# Autodesk Inventor assembly: ChainWheelSubAssembly
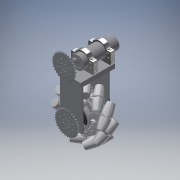
[picture p0: Inventor's stored thumbnail of the model, 180x180]
Saved by Autodesk Inventor 2017 (Build 210142000, 142)
## iProperties
Created: 2017-11-22
Part Number: ChainWheelSubAssembly
Document SubType Name: Assembly
Designer: User
Author: User
## Documents named in this file (9)
- C:\Robotics\CAD\2017-18_CAD\Prototypes\ChainWheelSubAssembly.iam
- C:\Robotics\CAD\COTSParts\Tetrix\tetrix-motor-mounts-1.snapshot.1\Tetrex 2pc motor mount.ipt
- C:\Robotics\CAD\COTSParts\Motors\Andymark 2964  NeveRest 40 Motor.ipt
- C:\Robotics\CAD\COTSParts\Actobotics\545 parts\545618 clamping hub.ipt
- C:\Robotics\CAD\COTSParts\Actobotics\615 parts\615114.ipt
- C:\Robotics\CAD\COTSParts\Vex\6inchMecanumRight217-2586-STEP\6inchMecanumRight217-2586.20121203.ipt
- C:\Robotics\CAD\COTSParts\Vex\VersaHub.5inchBore217-4009-STEP-20140807\VersaHub.5inchBore217-4009-STEP-20140807.ipt
- C:\Robotics\CAD\2017-18_CAD\Prototypes\Axle1.ipt
- C:\Robotics\CAD\2017-18_CAD\Prototypes\ChainWheelSubAssemblyMainConnector.ipt
## Components (13 placed, 8 different names)
1. Tetrex 2pc motor mount:1 — Mate:1, Mate:4, Flush:2, Mate:18, Mate:25, Flush:8
2. Tetrex 2pc motor mount:2 — Mate:2, Mate:3, Flush:2, Flush:7
3. Andymark 2964  NeveRest 40 Motor:1 — Mate:1, Mate:2, Mate:3, Mate:4, Mate:6, Mate:7, Flush:1, Mate:11
4. 545618 clamping hub:1 — Mate:6, Mate:8, Mate:9, Mate:10, Mate:11
5. 615114:1 — Mate:7, Flush:1, Mate:8, Mate:9, Mate:10, Flush:4
6. 615114:2 — Flush:4, Mate:18, Mate:19, Insert:1, Mate:21, Flush:5, Mate:22, Flush:6
7. 6inchMecanumRight217-2586.20121203:1 — Mate:12, Mate:13, Insert:1
8. VersaHub.5inchBore217-4009-STEP-20140807:1 — Mate:12, Mate:13, Mate:19, Insert:2, Mate:20, Mate:23, Insert:4
9. 545618 clamping hub:2 — Mate:21, Flush:5, Mate:22, Mate:24
10. 545618 clamping hub:3 — Insert:2, Mate:20, Insert:3
11. 545618 clamping hub:4 — Mate:23, Insert:3, Insert:4
12. Axle1:1 — Mate:24, Flush:6
13. ChainWheelSubAssemblyMainConnector:1 — Mate:25, Flush:7, Flush:8
## Relationships (31: Mate 20, Flush 7, Insert 4)
- Mate:1: Tetrex 2pc motor mount:1 ↔ Andymark 2964  NeveRest 40 Motor:1
- Mate:2: Tetrex 2pc motor mount:2 ↔ Andymark 2964  NeveRest 40 Motor:1
- Mate:3: Tetrex 2pc motor mount:2 ↔ Andymark 2964  NeveRest 40 Motor:1
- Mate:4: Tetrex 2pc motor mount:1 ↔ Andymark 2964  NeveRest 40 Motor:1
- Mate:6: Andymark 2964  NeveRest 40 Motor:1 ↔ 545618 clamping hub:1
- Mate:7: Andymark 2964  NeveRest 40 Motor:1 ↔ 615114:1
- Flush:1: Andymark 2964  NeveRest 40 Motor:1 ↔ 615114:1
- Mate:8: 545618 clamping hub:1 ↔ 615114:1
- Mate:9: 545618 clamping hub:1 ↔ 615114:1
- Mate:10: 545618 clamping hub:1 ↔ 615114:1
- Mate:11: Andymark 2964  NeveRest 40 Motor:1 ↔ 545618 clamping hub:1
- Flush:2: Tetrex 2pc motor mount:1 ↔ Tetrex 2pc motor mount:2
- Mate:12: 6inchMecanumRight217-2586.20121203:1 ↔ VersaHub.5inchBore217-4009-STEP-20140807:1
- Mate:13: 6inchMecanumRight217-2586.20121203:1 ↔ VersaHub.5inchBore217-4009-STEP-20140807:1
- Flush:4: 615114:1 ↔ 615114:2
- Mate:18 (76.2 mm): Tetrex 2pc motor mount:1 ↔ 615114:2
- Mate:19 (25.4 mm): 615114:2 ↔ VersaHub.5inchBore217-4009-STEP-20140807:1
- Insert:1: 615114:2 ↔ 6inchMecanumRight217-2586.20121203:1
- Insert:2: VersaHub.5inchBore217-4009-STEP-20140807:1 ↔ 545618 clamping hub:3
- Mate:20: VersaHub.5inchBore217-4009-STEP-20140807:1 ↔ 545618 clamping hub:3
- Mate:21: 615114:2 ↔ 545618 clamping hub:2
- Flush:5: 615114:2 ↔ 545618 clamping hub:2
- Mate:22: 615114:2 ↔ 545618 clamping hub:2
- Mate:23: VersaHub.5inchBore217-4009-STEP-20140807:1 ↔ 545618 clamping hub:4
- Insert:3: 545618 clamping hub:3 ↔ 545618 clamping hub:4
- Insert:4: VersaHub.5inchBore217-4009-STEP-20140807:1 ↔ 545618 clamping hub:4
- Mate:24: 545618 clamping hub:2 ↔ Axle1:1
- Flush:6: 615114:2 ↔ Axle1:1
- Mate:25: Tetrex 2pc motor mount:1 ↔ ChainWheelSubAssemblyMainConnector:1
- Flush:7: Tetrex 2pc motor mount:2 ↔ ChainWheelSubAssemblyMainConnector:1
- Flush:8: Tetrex 2pc motor mount:1 ↔ ChainWheelSubAssemblyMainConnector:1
